# Autodesk Inventor assembly: 4483T461_HIGH-STRENGTH BALL JOINT ROD END
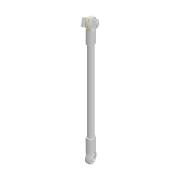
[picture p0: Inventor's stored thumbnail of the model, 180x180]
Saved by Autodesk Inventor 2021 (Build 250183000, 183)
## iProperties
Created: 2021-05-08
Part Number: 4483T461_HIGH-STRENGTH BALL JOINT ROD END
Document SubType Name: Assembly
Designer: Santiago Suárez
Author: Santiago Suárez
## Documents named in this file (6)
- C:\Users\Santiago Suárez\Documents\GitHub\Dis.-Mecatronico-E6\inventor proyecto\Biela.iam
- C:\Users\Santiago Suárez\Documents\GitHub\Dis.-Mecatronico-E6\inventor proyecto\Solid2.ipt
- C:\Users\Santiago Suárez\Documents\GitHub\Dis.-Mecatronico-E6\inventor proyecto\Solid1.ipt
- C:\Users\Santiago Suárez\Documents\GitHub\Dis.-Mecatronico-E6\inventor proyecto\BielaConexion.ipt
- C:\Users\Santiago Suárez\Documents\GitHub\Dis.-Mecatronico-E6\inventor proyecto\Eje.ipt
- C:\Users\Santiago Suárez\Documents\GitHub\Dis.-Mecatronico-E6\inventor proyecto\UnionMarco.ipt
## Components (7 placed, 5 different names)
1. BielaConexion:1 — Insert:1, Insert:2
2. Solid1:1 — Insert:1, Flush:1, Ball:1
3. Solid2:1 — Ball:1, Rigid:1
4. Solid1:2 — Insert:2, Flush:1, Ball:2
5. Solid2:2 — Ball:2
6. Eje:1 — Rigid:1, Rigid:2
7. UnionMarco:1 — Rigid:2
## Relationships (7: Insert 2, BallJoint 2, WeldJoint 2, Flush 1)
- Insert:1: BielaConexion:1 ↔ Solid1:1
- Insert:2: BielaConexion:1 ↔ Solid1:2
- Flush:1: Solid1:1 ↔ Solid1:2
- Ball:1: Solid1:1 ↔ Solid2:1
- Ball:2: Solid1:2 ↔ Solid2:2
- Rigid:1 [WeldJoint]: Solid2:1 ↔ Eje:1
- Rigid:2 [WeldJoint] (-3 mm): Eje:1 ↔ UnionMarco:1
